# Autodesk Inventor assembly: CPO-assembly
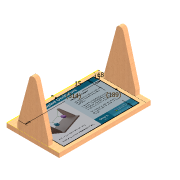
[picture p0: Inventor's stored thumbnail of the model, 180x180]
Saved by Autodesk Inventor 2020 (Build 240168000, 168)
## iProperties
Created: 2021-06-30
Part Number: CPO-assembly
Document SubType Name: Assembly
Designer: Aidan Lee
Author: Aidan Lee
## Documents named in this file (3)
- C:\Users\hobly\Dropbox\Aidan Lee\Mechanics_Walk\CoupledOscillators\CPO-assembly.iam
- C:\Users\hobly\Dropbox\Aidan Lee\Mechanics_Walk\CoupledOscillators\CPO-2-support.ipt
- C:\Users\hobly\Dropbox\Aidan Lee\Mechanics_Walk\CoupledOscillators\CPO-3-platform.ipt
## Components (3 placed, 2 different names)
1. CPO-2-support:1 — Mate:3, Mate:4, Flush:2
2. CPO-3-platform:1 — Mate:1, Flush:1, Mate:2, Mate:3, Mate:4, Flush:2
3. CPO-2-support:2 — Mate:1, Flush:1, Mate:2
## Relationships (6: Mate 4, Flush 2)
- Mate:1: CPO-3-platform:1 ↔ CPO-2-support:2
- Flush:1: CPO-3-platform:1 ↔ CPO-2-support:2
- Mate:2: CPO-3-platform:1 ↔ CPO-2-support:2
- Mate:3: CPO-2-support:1 ↔ CPO-3-platform:1
- Mate:4: CPO-2-support:1 ↔ CPO-3-platform:1
- Flush:2: CPO-2-support:1 ↔ CPO-3-platform:1
